# Autodesk Inventor assembly: Arm 2.0 Assembly
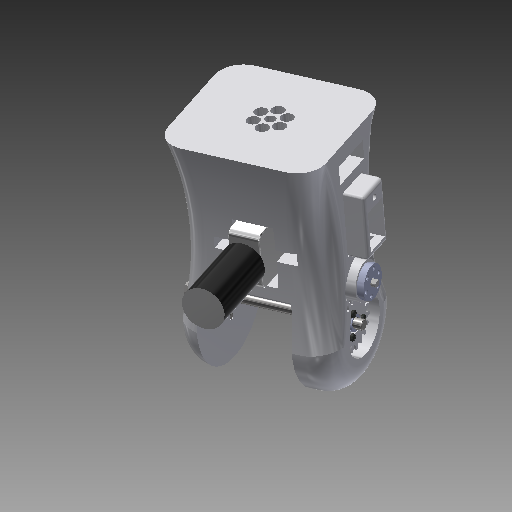
[picture p0: Inventor's stored thumbnail of the model, 512x512]
Saved by Autodesk Inventor 2017 (Build 210142000, 142)
## iProperties
Created: 2017-09-28
Part Number: Arm 2.0 Assembly
Document SubType Name: Assembly
Designer: Zach
Author: Zach
## Documents named in this file (16)
- C:\Users\Dell\Documents\GitHub\tr1\src\Body\Arm Assembly\Elbow Assembly\Elbow Assembly.iam
- C:\Users\Dell\Documents\GitHub\tr1\lib\22x8x8mm Bearing.ipt
- C:\Users\Dell\Documents\GitHub\tr1\src\Body\Arm Assembly\Elbow Assembly\Steel Rod 8mm x 110mm.ipt
- C:\Users\Dell\Documents\GitHub\tr1\src\Body\Arm Assembly\Elbow Assembly\AA014.ipt
- C:\Users\Dell\Documents\GitHub\tr1\lib\Content Center Files\R2017\en-US\ISO 4017(1)\ISO 4017 - M5 x 20 - ISO.ipt
- C:\Users\Dell\Documents\GitHub\tr1\src\Body\Arm Assembly\Elbow Assembly\AA010b.ipt
- C:\Users\Dell\Documents\GitHub\tr1\src\Body\Arm Assembly\Arm Assembly\Design Accelerator\Spur Gears10.iam
- C:\Users\Dell\Documents\GitHub\tr1\lib\Content Center Files\R2017\en-US\ISO 7045  H\ISO 7045 - M3 x 8 - 4.8 - H - ISO.ipt
- C:\Users\Dell\Documents\GitHub\tr1\lib\Content Center Files\R2017\en-US\ISO 4762(2)\ISO 4762 - M4 x 10ISO.ipt
- C:\Users\Dell\Documents\GitHub\tr1\lib\6mm Mounting Hub.ipt
- C:\Users\Dell\Documents\GitHub\tr1\lib\TSINY TS-42GZ495.ipt
- C:\Users\Dell\Documents\GitHub\tr1\lib\EMS22XXX-D28-LSX.ipt
- C:\Users\Dell\Documents\GitHub\tr1\src\Body\Arm Assembly\Elbow Assembly\AA053.ipt
- C:\Users\Dell\Documents\GitHub\tr1\src\Body\Arm Assembly\Elbow Assembly\AA055.ipt
- C:\Users\Dell\Documents\GitHub\tr1\src\Body\Arm Assembly\Elbow Assembly\AA057.ipt
- C:\Users\Dell\Documents\GitHub\tr1\src\Body\Arm Assembly\Elbow Assembly\AASG03a.ipt
## Components (22 placed, 15 different names)
1. AA010b:1 — Mate:620, Mate:621, Mate:626, Mate:628, Mate:630, Mate:642, Flush:20, Mate:648, Mate:650, Mate:948, Mate:1097, Mate:1098, Angle:21, Mate:1100, Mate:1101, Mate:1102, Mate:1126, Mate:1204, Mate:1258, Mate:1259, Mate:1260, Mate:1274, Mate:1277, Mate:1301, Mate:1302, Mate:1303, Mate:1304
2. AA014:2 — Mate:628, Mate:629, Mate:630, Mate:976, Mate:977, Mate:978, Mate:979, Mate:980, Mate:981
3. AA053:1 — Mate:1258, Mate:1259, Mate:1260
4. AA055:1 — Mate:1274, Mate:1277
5. AA057:2 — Mate:1300, Angle:1296, Mate:1301, Mate:1305, Mate:1306, Mate:1307
6. 22x8x8mm Bearing:3 — Mate:57, Mate:620, Mate:626
7. 22x8x8mm Bearing:4 — Mate:621, Mate:629, Mate:642
8. Steel Rod 8mm x 110mm:1 — Mate:57, Flush:20, Mate:649, Mate:1204, Mate:1283
9. TSINY TS-42GZ495:2 — Mate:1097, Mate:1098, Mate:1101, Mate:1102, Mate:1300, Angle:1296
10. 6mm Mounting Hub:7 — Mate:1185, Mate:1186, Mate:1188
11. 6mm Mounting Hub:11 — Mate:1283, Mate:1284
12. EMS22XXX-D28-LSX:3 — Angle:21, Mate:1100, Mate:1126, Mate:1185, Mate:1187
13. AASG03a — Mate:1305, Mate:1306, Mate:1307
14. AASG07 [sub-assembly] — Mate:648, Mate:649, Mate:650, Mate:958, Mate:959, Mate:960, Mate:961, Mate:962, Mate:963, Mate:1186, Mate:1187, Mate:1188, Mate:1284
15. ISO 7045 H M3 x 8 - 4.8 - H:24 — Mate:960, Mate:963
16. ISO 7045 H M3 x 8 - 4.8 - H:25 — Mate:958, Mate:962
17. ISO 7045 H M3 x 8 - 4.8 - H:26 — Mate:959, Mate:961
18. ISO 4762 M4 x 10:4 — Mate:948, Mate:1302
19. ISO 4017 M5 x 20:4 — Mate:978, Mate:980
20. ISO 4017 M5 x 20:5 — Mate:977, Mate:979
21. ISO 4017 M5 x 20:6 — Mate:976, Mate:981
22. ISO 4762 M4 x 10:5 — Mate:1303, Mate:1304
## Relationships (53: Mate 50, Angle 2, Flush 1)
- Mate:57: 22x8x8mm Bearing:3 ↔ Steel Rod 8mm x 110mm:1
- Mate:620: AA010b:1 ↔ 22x8x8mm Bearing:3
- Mate:621: AA010b:1 ↔ 22x8x8mm Bearing:4
- Flush:20 (0.5 mm): AA010b:1 ↔ Steel Rod 8mm x 110mm:1
- Mate:626: AA010b:1 ↔ 22x8x8mm Bearing:3
- Mate:628: AA010b:1 ↔ AA014:2
- Mate:629: AA014:2 ↔ 22x8x8mm Bearing:4
- Mate:630: AA010b:1 ↔ AA014:2
- Mate:642: AA010b:1 ↔ 22x8x8mm Bearing:4
- Mate:648: AA010b:1 ↔ AASG07
- Mate:649: Steel Rod 8mm x 110mm:1 ↔ AASG07
- Mate:650: AA010b:1 ↔ AASG07
- Mate:948: AA010b:1 ↔ ISO 4762 M4 x 10:4
- Mate:958: AASG07 ↔ ISO 7045 H M3 x 8 - 4.8 - H:25
- Mate:959: AASG07 ↔ ISO 7045 H M3 x 8 - 4.8 - H:26
- Mate:960: AASG07 ↔ ISO 7045 H M3 x 8 - 4.8 - H:24
- Mate:961: AASG07 ↔ ISO 7045 H M3 x 8 - 4.8 - H:26
- Mate:962: AASG07 ↔ ISO 7045 H M3 x 8 - 4.8 - H:25
- Mate:963: AASG07 ↔ ISO 7045 H M3 x 8 - 4.8 - H:24
- Mate:976: AA014:2 ↔ ISO 4017 M5 x 20:6
- Mate:977: AA014:2 ↔ ISO 4017 M5 x 20:5
- Mate:978: AA014:2 ↔ ISO 4017 M5 x 20:4
- Mate:979: AA014:2 ↔ ISO 4017 M5 x 20:5
- Mate:980: AA014:2 ↔ ISO 4017 M5 x 20:4
- Mate:981: AA014:2 ↔ ISO 4017 M5 x 20:6
- Mate:1097: AA010b:1 ↔ TSINY TS-42GZ495:2
- Mate:1098: AA010b:1 ↔ TSINY TS-42GZ495:2
- Angle:21 (0 deg): AA010b:1 ↔ EMS22XXX-D28-LSX:3
- Mate:1100: AA010b:1 ↔ EMS22XXX-D28-LSX:3
- Mate:1101: AA010b:1 ↔ TSINY TS-42GZ495:2
- Mate:1102: AA010b:1 ↔ TSINY TS-42GZ495:2
- Mate:1126: AA010b:1 ↔ EMS22XXX-D28-LSX:3
- Mate:1185: 6mm Mounting Hub:7 ↔ EMS22XXX-D28-LSX:3
- Mate:1186: 6mm Mounting Hub:7 ↔ AASG07
- Mate:1187: EMS22XXX-D28-LSX:3 ↔ AASG07
- Mate:1188: 6mm Mounting Hub:7 ↔ AASG07
- Mate:1204: AA010b:1 ↔ Steel Rod 8mm x 110mm:1
- Mate:1258: AA010b:1 ↔ AA053:1
- Mate:1259: AA010b:1 ↔ AA053:1
- Mate:1260 (0.5 mm): AA010b:1 ↔ AA053:1
- Mate:1274: AA010b:1 ↔ AA055:1
- Mate:1277: AA010b:1 ↔ AA055:1
- Mate:1283: Steel Rod 8mm x 110mm:1 ↔ 6mm Mounting Hub:11
- Mate:1284: 6mm Mounting Hub:11 ↔ AASG07
- Mate:1300: AA057:2 ↔ TSINY TS-42GZ495:2
- Angle:1296 (180 deg): AA057:2 ↔ TSINY TS-42GZ495:2
- Mate:1301: AA010b:1 ↔ AA057:2
- Mate:1302: AA010b:1 ↔ ISO 4762 M4 x 10:4
- Mate:1303: AA010b:1 ↔ ISO 4762 M4 x 10:5
- Mate:1304: AA010b:1 ↔ ISO 4762 M4 x 10:5
- Mate:1305: AA057:2 ↔ AASG03a
- Mate:1306: AA057:2 ↔ AASG03a
- Mate:1307: AA057:2 ↔ AASG03a
